# Autodesk Inventor assembly: Assembly
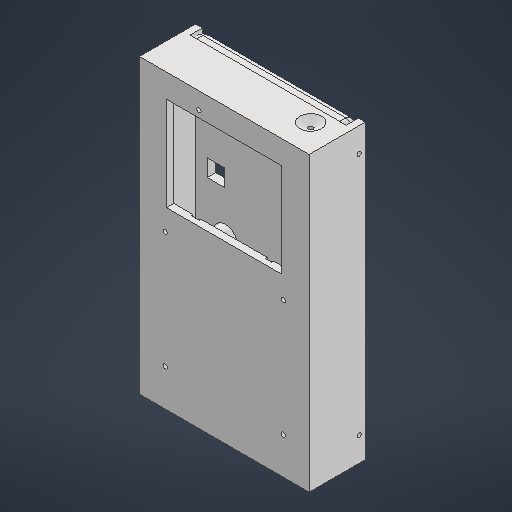
[picture p0: Inventor's stored thumbnail of the model, 512x512]
Saved by Autodesk Inventor 2027 (Build 310192000, 192)
## iProperties
Created: 2026-03-08
Part Number: Assembly
Document SubType Name: Assembly
Designer: kjedr
Author: kjedr
## Documents named in this file (5)
- C:\Users\kjedr\Documents\GitHub\ECE445-UIUC-Heterodyne\Chassis\Assembly.iam
- C:\Users\kjedr\Documents\GitHub\ECE445-UIUC-Heterodyne\Chassis\Top_Shell.ipt
- C:\Users\kjedr\Documents\GitHub\ECE445-UIUC-Heterodyne\Chassis\Bottom_Shell.ipt
- C:\Users\kjedr\Documents\GitHub\ECE445-UIUC-Heterodyne\Chassis\Dial.ipt
- C:\Users\kjedr\Documents\GitHub\ECE445-UIUC-Heterodyne\Chassis\freqDial1.ipt
## Components (4 placed, 4 different names)
1. Top_Shell:1 — Insert:1, Insert:2, Mate:1, Flush:1, Mate:2
2. Bottom_Shell:1 — Mate:1, Flush:1, Mate:2
3. Dial:2 — Insert:1
4. freqDial1:1 — Insert:2
## Relationships (5: Insert 2, Mate 2, Flush 1)
- Insert:1: Top_Shell:1 ↔ Dial:2
- Insert:2: Top_Shell:1 ↔ freqDial1:1
- Mate:1: Top_Shell:1 ↔ Bottom_Shell:1
- Flush:1: Top_Shell:1 ↔ Bottom_Shell:1
- Mate:2: Top_Shell:1 ↔ Bottom_Shell:1
